# Autodesk Inventor assembly: SlipRingAssy
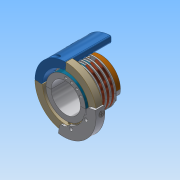
[picture p0: Inventor's stored thumbnail of the model, 180x180]
Saved by Autodesk Inventor 2017.3 (Build 213256000, 256)
## iProperties
Created: 2019-06-19
Part Number: SlipRingAssy
Document SubType Name: Assembly
Designer: Derek Wider
Author: Derek Wider
## Documents named in this file (9)
- G:\Projects\Submarine\Submarine-project\CAD\SlipRing\SlipRingAssy.iam
- G:\Projects\Submarine\Submarine-project\CAD\SlipRing\Core.ipt
- G:\Projects\Submarine\Submarine-project\CAD\SlipRing\CoreOpposite.ipt
- G:\Projects\Submarine\Submarine-project\CAD\SlipRing\BushingMount.ipt
- G:\Projects\Submarine\Submarine-project\CAD\SlipRing\ExtensionSpringSmall.ipt
- G:\Projects\Submarine\Submarine-project\CAD\SlipRing\BearingMount2.ipt
- G:\Projects\Submarine\Submarine-project\CAD\SlipRing\BearingMountBrace.ipt
- G:\Projects\Submarine\Submarine-project\CAD\common\screws\flatPlasticScrewSmall.ipt
- G:\Projects\Submarine\Submarine-project\CAD\SlipRing\CopperContact.ipt
## Components (12 placed, 8 different names)
1. Core:1 — Mate:1, Mate:2, Flush:1, Mate:3, Angle:1, Flush:2, Mate:15, Mate:16
2. CoreOpposite:1 — Mate:1, Mate:2, Flush:1, Mate:7, Mate:10
3. BushingMount:1 — Mate:3, Angle:1, Mate:6, Flush:2, Mate:8, Flush:3
4. ExtensionSpringSmall:1 — Mate:6
5. BearingMount2:1 — Mate:7, Mate:8, Flush:3, Mate:11, Mate:12, Mate:13, Mate:14
6. BearingMountBrace:1 — Mate:10, Mate:11, Mate:12, Tangent:1, Tangent:2
7. flatPlasticScrewSmall:1 — Mate:13, Tangent:1
8. flatPlasticScrewSmall:2 — Mate:14, Tangent:2
9. CopperContact:1 — Mate:15, Mate:16
10. CopperContact:2
11. CopperContact:3
12. CopperContact:4
## Component patterns: (4 elements, first: CopperContact:1)
## Relationships (19: Mate 13, Flush 3, Tangent 2, Angle 1)
- Mate:1: Core:1 ↔ CoreOpposite:1
- Mate:2: Core:1 ↔ CoreOpposite:1
- Flush:1: Core:1 ↔ CoreOpposite:1
- Mate:3: Core:1 ↔ BushingMount:1
- Angle:1 (0 deg): Core:1 ↔ BushingMount:1
- Mate:6: BushingMount:1 ↔ ExtensionSpringSmall:1
- Flush:2: Core:1 ↔ BushingMount:1
- Mate:7: CoreOpposite:1 ↔ BearingMount2:1
- Mate:8: BushingMount:1 ↔ BearingMount2:1
- Flush:3: BushingMount:1 ↔ BearingMount2:1
- Mate:10: CoreOpposite:1 ↔ BearingMountBrace:1
- Mate:11: BearingMount2:1 ↔ BearingMountBrace:1
- Mate:12: BearingMount2:1 ↔ BearingMountBrace:1
- Mate:13: BearingMount2:1 ↔ flatPlasticScrewSmall:1
- Tangent:1: BearingMountBrace:1 ↔ flatPlasticScrewSmall:1
- Mate:14: BearingMount2:1 ↔ flatPlasticScrewSmall:2
- Tangent:2: BearingMountBrace:1 ↔ flatPlasticScrewSmall:2
- Mate:15: Core:1 ↔ CopperContact:1
- Mate:16 (0.8255 mm): Core:1 ↔ CopperContact:1
